# Autodesk Inventor assembly: GFRP_T2_03
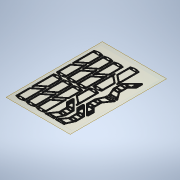
[picture p0: Inventor's stored thumbnail of the model, 180x180]
Saved by Autodesk Inventor 2020 (Build 240168000, 168)
## iProperties
Created: 2021-08-27
Part Number: GFRP_T2_03
Document SubType Name: Assembly
Designer: Masato
Author: Masato
## Documents named in this file (4)
- C:\Users\naoki\Documents\Inventor\CitBrains\git_clone\SUSTAINA_ver1_0\GFRP_2\SUSTAINA-OP\Cam\GFRP_T2_03.iam
- C:\Users\naoki\Documents\Inventor\CitBrains\git_clone\SUSTAINA_ver1_0\GFRP_2\SUSTAINA-OP\Cam\DisposableBoard.ipt
- C:\Users\naoki\Documents\Inventor\CitBrains\git_clone\SUSTAINA_ver1_0\GFRP_2\SUSTAINA-OP\UpperBody\Arm\UpperArm_side_frame.ipt
- C:\Users\naoki\Documents\Inventor\CitBrains\git_clone\SUSTAINA_ver1_0\GFRP_2\SUSTAINA-OP\UpperBody\Head\Head_side_frame.ipt
## Components (20 placed, 3 different names)
1. DisposableBoard:1 — メイト:2, メイト:1, フラッシュ:1, フラッシュ:2, フラッシュ:3, メイト:4, メイト:5, フラッシュ:4, メイト:11, メイト:12, メイト:13, メイト:15, メイト:17, メイト:20, メイト:21, フラッシュ:7
2. Head_side_frame:1 — メイト:12, 正接:2, メイト:23, フラッシュ:7, フラッシュ:8, メイト:24
3. Head_side_frame:2 — メイト:11, フラッシュ:8, メイト:24, メイト:26
4. UpperArm_side_frame:13 — メイト:15, 正接:2, メイト:25, メイト:27
5. UpperArm_side_frame:14 — メイト:21, 正接:3, 角度:1, メイト:28, 正接:4
6. UpperArm_side_frame:16 — メイト:13, メイト:19, メイト:27, 正接:3, 角度:1, 正接:4
7. Head_side_frame:3 — メイト:17, メイト:22, フラッシュ:6, メイト:26
8. Head_side_frame:4 — メイト:20, メイト:22, フラッシュ:6, メイト:28
9. UpperArm_side_frame:1 — メイト:5, フラッシュ:5, 正接:1
10. UpperArm_side_frame:2 — フラッシュ:3, メイト:4, フラッシュ:4, フラッシュ:5, 正接:1
11. UpperArm_side_frame:3
12. UpperArm_side_frame:4
13. UpperArm_side_frame:5
14. UpperArm_side_frame:6
15. UpperArm_side_frame:7
16. UpperArm_side_frame:8
17. UpperArm_side_frame:9 — メイト:25
18. UpperArm_side_frame:10 — メイト:23
19. UpperArm_side_frame:11 — メイト:19
20. UpperArm_side_frame:12
## Component patterns: (6 elements, first: UpperArm_side_frame:1 + UpperArm_side_frame:2)
## Relationships (32: Mate 19, Flush 8, Tangent 4, Angle 1)
- メイト:2 [Mate]: DisposableBoard:1
- メイト:1 [Mate]: DisposableBoard:1
- フラッシュ:1 [Flush]: DisposableBoard:1
- フラッシュ:2 [Flush]: DisposableBoard:1
- フラッシュ:3 [Flush] (2 mm): DisposableBoard:1 ↔ UpperArm_side_frame:2
- メイト:4 [Mate]: DisposableBoard:1 ↔ UpperArm_side_frame:2
- メイト:5 [Mate]: DisposableBoard:1 ↔ UpperArm_side_frame:1
- フラッシュ:4 [Flush] (2 mm): DisposableBoard:1 ↔ UpperArm_side_frame:2
- フラッシュ:5 [Flush]: UpperArm_side_frame:1 ↔ UpperArm_side_frame:2
- 正接:1 [Tangent] (2.5 mm): UpperArm_side_frame:1 ↔ UpperArm_side_frame:2
- メイト:11 [Mate]: DisposableBoard:1 ↔ Head_side_frame:2
- メイト:12 [Mate]: DisposableBoard:1 ↔ Head_side_frame:1
- メイト:13 [Mate]: DisposableBoard:1 ↔ UpperArm_side_frame:16
- メイト:15 [Mate]: DisposableBoard:1 ↔ UpperArm_side_frame:13
- メイト:17 [Mate]: DisposableBoard:1 ↔ Head_side_frame:3
- メイト:19 [Mate] (2.5 mm): UpperArm_side_frame:16 ↔ UpperArm_side_frame:11
- メイト:20 [Mate]: DisposableBoard:1 ↔ Head_side_frame:4
- メイト:21 [Mate]: DisposableBoard:1 ↔ UpperArm_side_frame:14
- メイト:22 [Mate] (2.5 mm): Head_side_frame:3 ↔ Head_side_frame:4
- フラッシュ:6 [Flush]: Head_side_frame:3 ↔ Head_side_frame:4
- 正接:2 [Tangent] (2.5 mm): Head_side_frame:1 ↔ UpperArm_side_frame:13
- メイト:23 [Mate] (2.5 mm): Head_side_frame:1 ↔ UpperArm_side_frame:10
- フラッシュ:7 [Flush] (2 mm): DisposableBoard:1 ↔ Head_side_frame:1
- フラッシュ:8 [Flush]: Head_side_frame:1 ↔ Head_side_frame:2
- メイト:24 [Mate] (3 mm): Head_side_frame:1 ↔ Head_side_frame:2
- メイト:25 [Mate] (2.5 mm): UpperArm_side_frame:13 ↔ UpperArm_side_frame:9
- メイト:26 [Mate] (2.5 mm): Head_side_frame:2 ↔ Head_side_frame:3
- メイト:27 [Mate] (2.5 mm): UpperArm_side_frame:13 ↔ UpperArm_side_frame:16
- 正接:3 [Tangent] (2.5 mm): UpperArm_side_frame:14 ↔ UpperArm_side_frame:16
- 角度:1 [Angle] (0 deg): UpperArm_side_frame:14 ↔ UpperArm_side_frame:16
- メイト:28 [Mate] (2.5 mm): UpperArm_side_frame:14 ↔ Head_side_frame:4
- 正接:4 [Tangent] (2.5 mm): UpperArm_side_frame:14 ↔ UpperArm_side_frame:16
